# Autodesk Inventor assembly: transmission
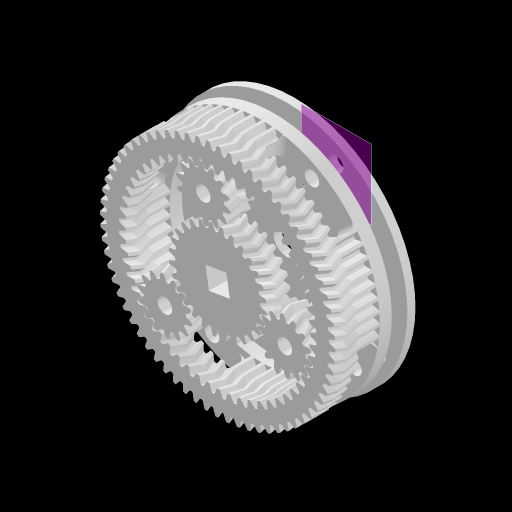
[picture p0: Inventor's stored thumbnail of the model, 512x512]
Saved by Autodesk Inventor 2024.1 (Build 281209000, 209)
## iProperties
Created: 2025-05-13
Part Number: transmission
Document SubType Name: Assembly
Designer: Teddy
Author: Teddy
## Documents named in this file (5)
- C:\Users\Teddy\OneDrive\Desktop\VEX-CAD-Inventor-1.4.0\pushBack\PushBackBot2\transmission.iam
- C:\Users\Teddy\OneDrive\Desktop\VEX-CAD-Inventor-1.4.0\2024-25 VexGame\GearBox\HerringBoneRingGear.ipt
- C:\Users\Teddy\OneDrive\Desktop\VEX-CAD-Inventor-1.4.0\2024-25 VexGame\GearBox\HerringBoneSunGear.ipt
- C:\Users\Teddy\OneDrive\Desktop\VEX-CAD-Inventor-1.4.0\2024-25 VexGame\GearBox\HerringBonePlanetGear.ipt
- C:\Users\Teddy\OneDrive\Desktop\cover.ipt
## Components (6 placed, 4 different names)
1. HerringBoneRingGear:1 — Insert:1, Flush:1, Flush:2
2. HerringBoneSunGear:1 — Insert:1
3. HerringBonePlanetGear:1
4. HerringBonePlanetGear:2
5. HerringBonePlanetGear:3
6. cover:1 — Flush:1, Flush:2
## Relationships (3: Flush 2, Insert 1)
- Insert:1: HerringBoneRingGear:1 ↔ HerringBoneSunGear:1
- Flush:1: HerringBoneRingGear:1 ↔ cover:1
- Flush:2: HerringBoneRingGear:1 ↔ cover:1
